# Autodesk Inventor assembly: arm
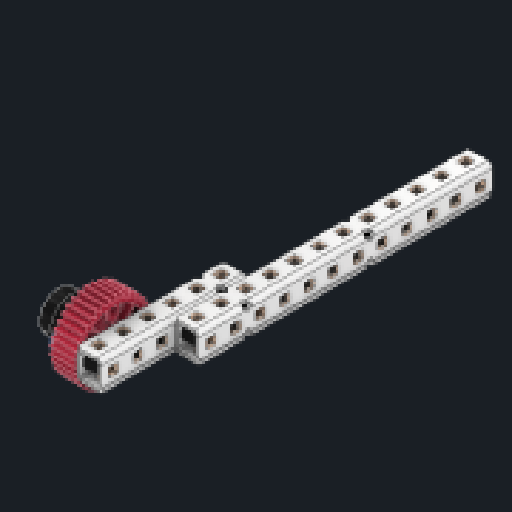
[picture p0: Inventor's stored thumbnail of the model, 512x512]
Saved by Autodesk Inventor 2024 (Build 280153000, 153)
## iProperties
Created: 2023-08-16
Part Number: arm
Document SubType Name: Assembly
Designer: avere
Author: avere
## Documents named in this file (11)
- D:\vex_robotics\hardware\cad\scrap_v0.1\catapult\arm.iam
- D:\vex_robotics\hardware\cad\VEX-CAD-Inventor-1.41\Motion\Spacers\Spacer Nylon .375 OD\NSpacer .375 OD x .375.ipt
- D:\vex_robotics\hardware\cad\VEX-CAD-Inventor-1.41\Motion\Spacers\Spacer Nylon .375 OD.ipt
- D:\vex_robotics\hardware\cad\VEX-CAD-Inventor-1.41\Motion\Gears\HS Gear\HS 36T Gear, No Insert.iam
- D:\vex_robotics\hardware\cad\VEX-CAD-Inventor-1.41\Motion\Gears\HS Gear.iam
- D:\vex_robotics\hardware\cad\VEX-CAD-Inventor-1.41\Structure\Angle\Aluminum 1x1\Alu Angle 1x1x6.ipt
- D:\vex_robotics\hardware\cad\VEX-CAD-Inventor-1.41\Motion\Shaft HS\HS Shaft Collar.ipt
- D:\vex_robotics\hardware\cad\VEX-CAD-Inventor-1.41\Motion\Shaft HS\HS Spacer\HSpacer .1250.ipt
- D:\vex_robotics\hardware\cad\VEX-CAD-Inventor-1.41\Motion\Shaft HS\HS Spacer.ipt
- D:\vex_robotics\hardware\cad\VEX-CAD-Inventor-1.41\Structure\Hardware\Nut Hex.ipt
- D:\vex_robotics\hardware\cad\VEX-CAD-Inventor-1.41\Structure\Angle\Aluminum 1x1\Alu Angle 1x1x12.ipt
## Components (14 placed, 7 different names)
1. HS 36T Gear, No Insert:1 [sub-assembly] — Insert:11, Mate:2, Insert:14, Insert:15, Insert:16
2. Alu Angle 1x1x6:1 — Insert:7, Insert:9, Insert:11, Mate:2, Insert:17
3. Alu Angle 1x1x6:2 — Insert:8, Insert:10, Insert:18, Mate:3
4. NSpacer .375 OD x .375:3 — Insert:7, Insert:8
5. NSpacer .375 OD x .375:4 — Insert:9, Insert:10
6. HS Shaft Collar:1
7. HSpacer .1250:1 — Insert:14
8. Nut Hex:1 — Insert:16
9. Nut Hex:2 — Insert:15
10. NSpacer .375 OD x .375:5 — Insert:17
11. Alu Angle 1x1x12:1 — Insert:21, Mate:4
12. Alu Angle 1x1x12:2 — Insert:18, Mate:3, Insert:19, Insert:20
13. NSpacer .375 OD x .375:6 — Insert:20, Mate:4
14. NSpacer .375 OD x .375:7 — Insert:19, Insert:21
## Relationships (17: Insert 14, Mate 3)
- Insert:7: Alu Angle 1x1x6:1 ↔ NSpacer .375 OD x .375:3
- Insert:8: Alu Angle 1x1x6:2 ↔ NSpacer .375 OD x .375:3
- Insert:9: Alu Angle 1x1x6:1 ↔ NSpacer .375 OD x .375:4
- Insert:10: Alu Angle 1x1x6:2 ↔ NSpacer .375 OD x .375:4
- Insert:11: HS 36T Gear, No Insert:1 ↔ Alu Angle 1x1x6:1
- Mate:2: HS 36T Gear, No Insert:1 ↔ Alu Angle 1x1x6:1
- [Insert]: HS Shaft Collar:1 ↔ HSpacer .1250:1
- Insert:14: HS 36T Gear, No Insert:1 ↔ HSpacer .1250:1
- Insert:15: HS 36T Gear, No Insert:1 ↔ Nut Hex:2
- Insert:16: HS 36T Gear, No Insert:1 ↔ Nut Hex:1
- Insert:17: Alu Angle 1x1x6:1 ↔ NSpacer .375 OD x .375:5
- Insert:18: Alu Angle 1x1x6:2 ↔ Alu Angle 1x1x12:2
- Mate:3: Alu Angle 1x1x6:2 ↔ Alu Angle 1x1x12:2
- Insert:19: Alu Angle 1x1x12:2 ↔ NSpacer .375 OD x .375:7
- Insert:20: Alu Angle 1x1x12:2 ↔ NSpacer .375 OD x .375:6
- Insert:21: Alu Angle 1x1x12:1 ↔ NSpacer .375 OD x .375:7
- Mate:4: Alu Angle 1x1x12:1 ↔ NSpacer .375 OD x .375:6
